# Autodesk Inventor assembly: Assembly2
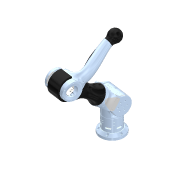
[picture p0: Inventor's stored thumbnail of the model, 180x180]
Saved by Autodesk Inventor 2021 (Build 250183000, 183)
## iProperties
Created: 2020-08-06
Part Number: Assembly2
Document SubType Name: Assembly
Designer: Derm
Mass: 2850.65 g
Surface Area: 9470.08 cm^2
Volume: 2711.95 cm^3
Density: 1.05114 g/cm^3
Author: Derm
## Documents named in this file (15)
- C:\Users\Derm\roboticArm\hardware\v9\Assembly2.iam
- C:\Users\Derm\roboticArm\hardware\v9\j0.iam
- C:\Users\Derm\roboticArm\hardware\v9\j1.iam
- C:\Users\Derm\roboticArm\hardware\v9\upperArmMain.ipt
- C:\Users\Derm\roboticArm\hardware\v9\upperArmMainSidePlate.ipt
- C:\Users\Derm\roboticArm\hardware\v9\2020 Aluminium Extrusion T-Slot.ipt
- C:\Users\Derm\roboticArm\hardware\v9\j1Flange.ipt
- C:\Users\Derm\roboticArm\hardware\v9\upperArmMid.ipt
- C:\Users\Derm\roboticArm\hardware\v9\j2.iam
- C:\Users\Derm\roboticArm\hardware\v9\elbowMain.ipt
- C:\Users\Derm\roboticArm\hardware\v9\upperArmMainCover.ipt
- C:\Users\Derm\roboticArm\hardware\v9\upperArmMidV2.ipt
- C:\Users\Derm\roboticArm\hardware\v9\elbowMainV2.ipt
- C:\Users\Derm\roboticArm\hardware\v9\endEffector.ipt
- C:\Users\Derm\roboticArm\hardware\v9\upperArmSidePlateSupport.ipt
## Components (16 placed, 14 different names)
1. j0:1 [sub-assembly] — Mate:1, Mate:2, Mate:3, Mate:6
2. j1:1 [sub-assembly] — Mate:2, Mate:3, Mate:6, Mate:7, Mate:8, Mate:11, Mate:14, Mate:15
3. upperArmMain:1 — Mate:7, Mate:8, Mate:10, Mate:12, Angle:2, Mate:13, Flush:1, Mate:19, Mate:22, Mate:27, Flush:2, Angle:3, Flush:3, Flush:4, Flush:5, Mate:34, Mate:35
4. upperArmMainSidePlate:1 — Mate:10, Mate:11, Mate:19, Mate:42, Mate:43, Mate:44
5. 2020 Aluminium Extrusion T-Slot:1 — Mate:12, Angle:2, Mate:13, Mate:23, Mate:24, Mate:26, Mate:30
6. j1Flange:1 — Mate:14, Mate:15
7. upperArmMid:1 — Flush:1, Mate:22, Mate:23
8. elbowMain:1 — Mate:24, Mate:26, Mate:27, Mate:28, Mate:29
9. upperArmMainSidePlate:2
10. j2:1 [sub-assembly] — Mate:28, Mate:29, Mate:32, Angle:4, Mate:40, Mate:41, Flush:6
11. upperArmMainCover:1 — Flush:2, Mate:34, Mate:35
12. upperArmMidV2:1 — Flush:3, Flush:4, Flush:5, Mate:33, Mate:38, Mate:39
13. elbowMainV2:1 — Mate:30, Mate:32, Mate:33, Mate:38, Mate:39
14. 2020 Aluminium Extrusion T-Slot:2
15. endEffector:1 — Angle:4, Mate:40, Mate:41, Flush:6
16. upperArmSidePlateSupport:1 — Mate:42, Mate:43, Mate:44
## Relationships (41: Mate 32, Flush 6, Angle 3)
- Mate:1: j0:1
- Mate:2: j0:1 ↔ j1:1
- Mate:3: j0:1 ↔ j1:1
- Mate:6: j0:1 ↔ j1:1
- Mate:7: j1:1 ↔ upperArmMain:1
- Mate:8: j1:1 ↔ upperArmMain:1
- Mate:10: upperArmMain:1 ↔ upperArmMainSidePlate:1
- Mate:11: j1:1 ↔ upperArmMainSidePlate:1
- Mate:12: upperArmMain:1 ↔ 2020 Aluminium Extrusion T-Slot:1
- Angle:2 (0 deg): upperArmMain:1 ↔ 2020 Aluminium Extrusion T-Slot:1
- Mate:13: upperArmMain:1 ↔ 2020 Aluminium Extrusion T-Slot:1
- Mate:14: j1:1 ↔ j1Flange:1
- Mate:15: j1:1 ↔ j1Flange:1
- Flush:1: upperArmMain:1 ↔ upperArmMid:1
- Mate:19: upperArmMain:1 ↔ upperArmMainSidePlate:1
- Mate:22: upperArmMain:1 ↔ upperArmMid:1
- Mate:23: 2020 Aluminium Extrusion T-Slot:1 ↔ upperArmMid:1
- Mate:24: 2020 Aluminium Extrusion T-Slot:1 ↔ elbowMain:1
- Mate:26: 2020 Aluminium Extrusion T-Slot:1 ↔ elbowMain:1
- Mate:27: upperArmMain:1 ↔ elbowMain:1
- Mate:28: elbowMain:1 ↔ j2:1
- Flush:2: upperArmMain:1 ↔ upperArmMainCover:1
- Mate:29: elbowMain:1 ↔ j2:1
- Angle:3 (0 deg): upperArmMain:1
- Flush:3: upperArmMain:1 ↔ upperArmMidV2:1
- Flush:4 (120.65 mm): upperArmMain:1 ↔ upperArmMidV2:1
- Mate:30: 2020 Aluminium Extrusion T-Slot:1 ↔ elbowMainV2:1
- Mate:32: j2:1 ↔ elbowMainV2:1
- Flush:5 (50.8 mm): upperArmMain:1 ↔ upperArmMidV2:1
- Mate:33: upperArmMidV2:1 ↔ elbowMainV2:1
- Mate:34: upperArmMain:1 ↔ upperArmMainCover:1
- Mate:35: upperArmMain:1 ↔ upperArmMainCover:1
- Angle:4 (0 deg): j2:1 ↔ endEffector:1
- Mate:38: upperArmMidV2:1 ↔ elbowMainV2:1
- Mate:39: upperArmMidV2:1 ↔ elbowMainV2:1
- Mate:40: j2:1 ↔ endEffector:1
- Mate:41: j2:1 ↔ endEffector:1
- Flush:6: j2:1 ↔ endEffector:1
- Mate:42: upperArmMainSidePlate:1 ↔ upperArmSidePlateSupport:1
- Mate:43: upperArmMainSidePlate:1 ↔ upperArmSidePlateSupport:1
- Mate:44: upperArmMainSidePlate:1 ↔ upperArmSidePlateSupport:1
